# Autodesk Inventor assembly: FrameV2
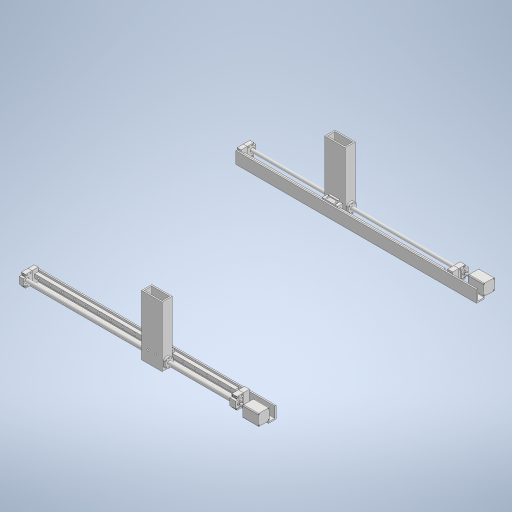
[picture p0: Inventor's stored thumbnail of the model, 512x512]
Saved by Autodesk Inventor 2023 (Build 270158000, 158)
## iProperties
Created: 2022-05-01
Part Number: FrameV2
Document SubType Name: Assembly
Designer: plebbb
Author: plebbb
## Documents named in this file (13)
- D:\Users\plebbb\Desktop\CNC_Project\FrameV2.iam
- D:\Users\plebbb\Desktop\CNC_Project\HGW20CC_Rail_800mm.ipt
- D:\Users\plebbb\Desktop\CNC_Project\HGW20CC_Slider.ipt
- D:\Users\plebbb\Desktop\CNC_Project\SFU1605_800mm.ipt
- D:\Users\plebbb\Desktop\CNC_Project\SFU1605_Nut.ipt
- D:\Users\plebbb\Desktop\CNC_Project\BF12.ipt
- D:\Users\plebbb\Desktop\CNC_Project\BK12.ipt
- D:\Users\plebbb\Desktop\CNC_Project\VERTICALTUBE.ipt
- D:\Users\plebbb\Desktop\CNC_Project\Steel_L_Bracket.ipt
- D:\Users\plebbb\Desktop\CNC_Project\BF12_Spacer.ipt
- D:\Users\plebbb\Desktop\CNC_Project\BK12_Spacer.ipt
- D:\Users\plebbb\Desktop\CNC_Project\Nema23.ipt
- D:\Users\plebbb\Desktop\CNC_Project\VERTICALTUBE_Reverse.ipt
## Components (22 placed, 12 different names)
1. VERTICALTUBE_Reverse:1 — Mate:64, Mate:65, Mate:66, Mate:72, Mate:76
2. Steel_L_Bracket:2 — Flush:25, Mate:48, Mate:52, Flush:52, Angle:3, Flush:54, Flush:55, Mate:67, Flush:56, Flush:57, Mate:77
3. HGW20CC_Rail_800mm:2 — Flush:25, Mate:48, Mate:59, Mate:60, Mate:75
4. BK12_Spacer:2 — Mate:52, Flush:52, Mate:56, Mate:57, Mate:58
5. BF12:2 — Mate:62, Mate:68, Mate:69, Mate:70, Mate:72
6. BK12:2 — Mate:56, Mate:57, Mate:58, Mate:61, Flush:53
7. SFU1605_800mm:2 — Mate:61, Flush:53, Mate:62, Mate:63, Mate:64, Mate:71, Mate:73, Mate:74
8. HGW20CC_Slider:3 — Mate:59, Mate:60, Mate:76
9. SFU1605_Nut:2 — Mate:63, Angle:3, Mate:65, Mate:66, Mate:71
10. BF12_Spacer:2 — Flush:54, Flush:55, Mate:67, Mate:68, Mate:69, Mate:70, Mate:75
11. Nema23:2 — Mate:73, Mate:74
12. HGW20CC_Rail_800mm:1 — Mate:3, Mate:4, Flush:1, Flush:21, Mate:35, Mate:38
13. SFU1605_800mm:1 — Mate:9, Mate:16, Flush:19, Mate:17, Mate:18, Mate:32, Mate:44, Mate:46, Mate:47
14. SFU1605_Nut:1 — Mate:9, Mate:33, Mate:34, Mate:44
15. HGW20CC_Slider:2 — Mate:3, Mate:4, Flush:1, Mate:25, Mate:30, Mate:31
16. BF12:1 — Mate:17, Mate:18, Angle:1, Mate:37, Mate:45
17. BK12:1 — Mate:16, Flush:19, Angle:2, Mate:40, Mate:41
18. VERTICALTUBE:1 — Mate:25, Mate:30, Mate:31, Mate:32, Mate:33, Mate:34, Mate:45
19. Steel_L_Bracket:1 — Flush:21, Mate:35, Angle:1, Mate:36, Flush:22, Flush:23, Angle:2, Mate:39, Flush:24, Mate:42, Mate:43, Flush:56, Flush:57, Mate:77
20. BF12_Spacer:1 — Mate:36, Flush:22, Flush:23, Mate:37, Mate:38
21. BK12_Spacer:1 — Mate:39, Flush:24, Mate:40, Mate:41
22. Nema23:1 — Mate:46, Mate:47
## Relationships (65: Mate 49, Flush 13, Angle 3)
- Mate:3: HGW20CC_Rail_800mm:1 ↔ HGW20CC_Slider:2
- Mate:4: HGW20CC_Rail_800mm:1 ↔ HGW20CC_Slider:2
- Mate:9: SFU1605_800mm:1 ↔ SFU1605_Nut:1
- Flush:1: HGW20CC_Rail_800mm:1 ↔ HGW20CC_Slider:2
- Mate:16: SFU1605_800mm:1 ↔ BK12:1
- Flush:19: SFU1605_800mm:1 ↔ BK12:1
- Mate:17: SFU1605_800mm:1 ↔ BF12:1
- Mate:18: SFU1605_800mm:1 ↔ BF12:1
- Mate:25: HGW20CC_Slider:2 ↔ VERTICALTUBE:1
- Mate:30: HGW20CC_Slider:2 ↔ VERTICALTUBE:1
- Mate:31: HGW20CC_Slider:2 ↔ VERTICALTUBE:1
- Mate:32: SFU1605_800mm:1 ↔ VERTICALTUBE:1
- Mate:33: SFU1605_Nut:1 ↔ VERTICALTUBE:1
- Mate:34: SFU1605_Nut:1 ↔ VERTICALTUBE:1
- Flush:21 (10 mm): HGW20CC_Rail_800mm:1 ↔ Steel_L_Bracket:1
- Mate:35: HGW20CC_Rail_800mm:1 ↔ Steel_L_Bracket:1
- Angle:1 (0 deg): BF12:1 ↔ Steel_L_Bracket:1
- Mate:36: Steel_L_Bracket:1 ↔ BF12_Spacer:1
- Flush:22: Steel_L_Bracket:1 ↔ BF12_Spacer:1
- Flush:23 (-10 mm): Steel_L_Bracket:1 ↔ BF12_Spacer:1
- Mate:37: BF12:1 ↔ BF12_Spacer:1
- Angle:2 (0 deg): BK12:1 ↔ Steel_L_Bracket:1
- Mate:38: HGW20CC_Rail_800mm:1 ↔ BF12_Spacer:1
- Mate:39: Steel_L_Bracket:1 ↔ BK12_Spacer:1
- Flush:24 (-10 mm): Steel_L_Bracket:1 ↔ BK12_Spacer:1
- Mate:40: BK12:1 ↔ BK12_Spacer:1
- Mate:41: BK12:1 ↔ BK12_Spacer:1
- Mate:42: Steel_L_Bracket:1
- Mate:43: Steel_L_Bracket:1
- Mate:44: SFU1605_800mm:1 ↔ SFU1605_Nut:1
- Mate:45: BF12:1 ↔ VERTICALTUBE:1
- Mate:46: SFU1605_800mm:1 ↔ Nema23:1
- Mate:47: SFU1605_800mm:1 ↔ Nema23:1
- Flush:25 (10 mm): Steel_L_Bracket:2 ↔ HGW20CC_Rail_800mm:2
- Mate:48: Steel_L_Bracket:2 ↔ HGW20CC_Rail_800mm:2
- Mate:52: Steel_L_Bracket:2 ↔ BK12_Spacer:2
- Flush:52 (10 mm): Steel_L_Bracket:2 ↔ BK12_Spacer:2
- Mate:56: BK12_Spacer:2 ↔ BK12:2
- Mate:57: BK12_Spacer:2 ↔ BK12:2
- Mate:58: BK12_Spacer:2 ↔ BK12:2
- Mate:59: HGW20CC_Rail_800mm:2 ↔ HGW20CC_Slider:3
- Mate:60: HGW20CC_Rail_800mm:2 ↔ HGW20CC_Slider:3
- Mate:61: BK12:2 ↔ SFU1605_800mm:2
- Flush:53: BK12:2 ↔ SFU1605_800mm:2
- Mate:62: BF12:2 ↔ SFU1605_800mm:2
- Mate:63: SFU1605_800mm:2 ↔ SFU1605_Nut:2
- Mate:64: VERTICALTUBE_Reverse:1 ↔ SFU1605_800mm:2
- Angle:3 (0 deg): Steel_L_Bracket:2 ↔ SFU1605_Nut:2
- Mate:65: VERTICALTUBE_Reverse:1 ↔ SFU1605_Nut:2
- Mate:66: VERTICALTUBE_Reverse:1 ↔ SFU1605_Nut:2
- Flush:54 (-10 mm): Steel_L_Bracket:2 ↔ BF12_Spacer:2
- Flush:55: Steel_L_Bracket:2 ↔ BF12_Spacer:2
- Mate:67: Steel_L_Bracket:2 ↔ BF12_Spacer:2
- Mate:68: BF12:2 ↔ BF12_Spacer:2
- Mate:69: BF12:2 ↔ BF12_Spacer:2
- Mate:70: BF12:2 ↔ BF12_Spacer:2
- Mate:71: SFU1605_800mm:2 ↔ SFU1605_Nut:2
- Mate:72: VERTICALTUBE_Reverse:1 ↔ BF12:2
- Mate:73: SFU1605_800mm:2 ↔ Nema23:2
- Mate:74: SFU1605_800mm:2 ↔ Nema23:2
- Flush:56: Steel_L_Bracket:2 ↔ Steel_L_Bracket:1
- Mate:75: HGW20CC_Rail_800mm:2 ↔ BF12_Spacer:2
- Flush:57: Steel_L_Bracket:2 ↔ Steel_L_Bracket:1
- Mate:76: VERTICALTUBE_Reverse:1 ↔ HGW20CC_Slider:3
- Mate:77 (1000 mm): Steel_L_Bracket:2 ↔ Steel_L_Bracket:1
